# Autodesk Inventor assembly: Main_assssembly
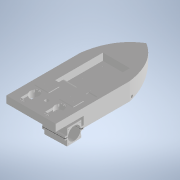
[picture p0: Inventor's stored thumbnail of the model, 180x180]
Saved by Autodesk Inventor 2020.1 (Build 241239000, 239)
## iProperties
Created: 2022-02-07
Part Number: Main_assssembly
Document SubType Name: Assembly
Designer: OEM
Author: OEM
## Documents named in this file (9)
- D:\Studia\Bobr\Repo\CAD\Main_assssembly.iam
- D:\Studia\Bobr\Repo\CAD\MainBody.ipt
- D:\Studia\Bobr\Repo\CAD\connector_sleeve.ipt
- D:\Studia\Bobr\Repo\CAD\engine_cup.ipt
- D:\Studia\Bobr\Repo\CAD\engine_lid.ipt
- D:\Studia\Bobr\Repo\CAD\engine_sleeve_up.ipt
- D:\Studia\Bobr\Repo\CAD\Bought_parts\Seal.ipt
- D:\Studia\Bobr\Repo\CAD\engine_sleeve_down.ipt
- D:\Studia\Bobr\Repo\CAD\Bought_parts\motor_subsitude.ipt
## Components (9 placed, 8 different names)
1. MainBody:2 — Rotational:1, Mate:6
2. connector_sleeve:1 — Rotational:1, Mate:5
3. engine_cup:1 — Rigid:5, Mate:7, Mate:8, Mate:9
4. engine_lid:1
5. engine_sleeve_up:1 — Mate:5, Mate:6, Rigid:1, Rigid:3, Rigid:5
6. Seal:1 — Rigid:3
7. Seal:2 — Rigid:1, Rigid:4
8. engine_sleeve_down:1 — Rigid:4
9. motor_subsitude:1 — Mate:7, Mate:8, Mate:9
## Relationships (10: Mate 5, WeldJoint 4, RevoluteJoint 1)
- Rotational:1 [RevoluteJoint]: MainBody:2 ↔ connector_sleeve:1
- Mate:5: connector_sleeve:1 ↔ engine_sleeve_up:1
- Mate:6: MainBody:2 ↔ engine_sleeve_up:1
- Rigid:1 [WeldJoint]: engine_sleeve_up:1 ↔ Seal:2
- Rigid:3 [WeldJoint]: engine_sleeve_up:1 ↔ Seal:1
- Rigid:4 [WeldJoint]: Seal:2 ↔ engine_sleeve_down:1
- Rigid:5 [WeldJoint]: engine_cup:1 ↔ engine_sleeve_up:1
- Mate:7: engine_cup:1 ↔ motor_subsitude:1
- Mate:8: engine_cup:1 ↔ motor_subsitude:1
- Mate:9: engine_cup:1 ↔ motor_subsitude:1
